# Autodesk Inventor assembly: WCP-0235
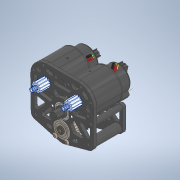
[picture p0: Inventor's stored thumbnail of the model, 180x180]
Saved by Autodesk Inventor 2020 (Build 240168000, 168)
## iProperties
Created: 2019-12-21
Part Number: WCP-0235
Description: STEP AP214
Document SubType Name: Assembly
Designer: 23kaltomare
Mass: 1814.37 g
Surface Area: 1714.71 cm^2
Volume: 577.017 cm^3
Sending System: SolidWorks 2018
Preprocessor: SwSTEP 2.0
Title: WCP-0235 Rev1 - WCP SS Flipped Gearbox (SingleSpeed, 2 Stages).STEP
Revision Number: ANY
## Documents named in this file (19)
- T:\EIT\2022 Rapid React\COMMON PARTS\GEARBOXES\WCP-0235.iam
- T:\EIT\2022 Rapid React\COMMON PARTS\GEARBOXES\WCP-0235-001 Rev1.ipt
- T:\EIT\2022 Rapid React\COMMON PARTS\GEARBOXES\WCP-0235-002 Rev1.ipt
- T:\EIT\2022 Rapid React\COMMON PARTS\GEARBOXES\12T_20dp_Falcon_Motor_217-6919.ipt
- T:\EIT\2022 Rapid React\COMMON PARTS\GEARBOXES\60T_20dp_hex_0_500_217-3574.ipt
- T:\EIT\2022 Rapid React\COMMON PARTS\GEARBOXES\thunderhex_flanged_217-4006.ipt
- T:\EIT\2022 Rapid React\COMMON PARTS\GEARBOXES\BHCS_10-32_0_250_91255A261_91255A261.ipt
- T:\EIT\2022 Rapid React\COMMON PARTS\GEARBOXES\22T_steel_20dp_hex_0_500_217-5463.ipt
- T:\EIT\2022 Rapid React\COMMON PARTS\GEARBOXES\16T_#25_500_hex_hubbed_sprocket_217-2642.ipt
- T:\EIT\2022 Rapid React\COMMON PARTS\GEARBOXES\375ID_875OD_flanged_217-2733.ipt
- T:\EIT\2022 Rapid React\COMMON PARTS\GEARBOXES\WCP-0155-012 Rev1.ipt
- T:\EIT\2022 Rapid React\COMMON PARTS\GEARBOXES\500ID_1_125OD_flanged_217_2731.ipt
- T:\EIT\2022 Rapid React\COMMON PARTS\GEARBOXES\WCP-0235-003 Rev1.ipt
- T:\EIT\2022 Rapid React\COMMON PARTS\GEARBOXES\26T_steel_20dp_hex_0_500_217-5466.ipt
- T:\EIT\2022 Rapid React\COMMON PARTS\GEARBOXES\0_125_L_500_hex_spacer_217-2758.ipt
- T:\EIT\2022 Rapid React\COMMON PARTS\GEARBOXES\WCP-0207 Rev1.ipt
- T:\EIT\2022 Rapid React\COMMON PARTS\GEARBOXES\WCP-0235-004 Rev1.ipt
- T:\EIT\2022 Rapid React\COMMON PARTS\GEARBOXES\217-6515_Falcon_500_Default_As Machined_.ipt
- T:\EIT\2022 Rapid React\DRIVE BASE\SPACERS\DB-SP-004.ipt
## Components (24 placed, 24 different names)
1. WCP-0235-001 Rev1_1
2. WCP-0235-002 Rev1_2
3. 12T_20dp_Falcon_Motor_217-6919_3
4. 12T_20dp_Falcon_Motor_217-6919_4
5. 60T_20dp_hex_0_500_217-3574_5
6. thunderhex_flanged_217-4006_6
7. BHCS_10-32_0_250_91255A261_91255A261_7
8. 22T_steel_20dp_hex_0_500_217-5463_8
9. 16T_#25_500_hex_hubbed_sprocket_217-2642_10 — Mate:1, Angle:1, Mate:3, Mate:4
10. 16T_#25_500_hex_hubbed_sprocket_217-2642_11 — Mate:2, Angle:2, Mate:4
11. 375ID_875OD_flanged_217-2733_12
12. WCP-0155-012 Rev1_13 — Mate:1, Angle:1, Mate:2, Angle:2
13. 500ID_1_125OD_flanged_217_2731_14
14. WCP-0235-003 Rev1_15
15. 26T_steel_20dp_hex_0_500_217-5466_16 — Mate:3, Insert:1
16. 0_125_L_500_hex_spacer_217-2758_17
17. BHCS_10-32_0_250_91255A261_91255A261_18
18. WCP-0207 Rev1_19
19. WCP-0207 Rev1_20
20. WCP-0235-004 Rev1_21
21. WCP-0235-004 Rev1_22
22. 217-6515_Falcon_500_Default<As Machined>_23
23. 217-6515_Falcon_500_Default<As Machined>_24
24. DB-SP-004:1 — Insert:1
## Relationships (7: Mate 4, Angle 2, Insert 1)
- Mate:1: 16T_#25_500_hex_hubbed_sprocket_217-2642_10 ↔ WCP-0155-012 Rev1_13
- Angle:1 (0 deg): 16T_#25_500_hex_hubbed_sprocket_217-2642_10 ↔ WCP-0155-012 Rev1_13
- Mate:2: 16T_#25_500_hex_hubbed_sprocket_217-2642_11 ↔ WCP-0155-012 Rev1_13
- Angle:2 (0 deg): 16T_#25_500_hex_hubbed_sprocket_217-2642_11 ↔ WCP-0155-012 Rev1_13
- Mate:3 (1.1176 mm): 16T_#25_500_hex_hubbed_sprocket_217-2642_10 ↔ 26T_steel_20dp_hex_0_500_217-5466_16
- Mate:4: 16T_#25_500_hex_hubbed_sprocket_217-2642_10 ↔ 16T_#25_500_hex_hubbed_sprocket_217-2642_11
- Insert:1: 26T_steel_20dp_hex_0_500_217-5466_16 ↔ DB-SP-004:1
